# Autodesk Inventor assembly: GarageAndBracket3inchPvcPipeV02
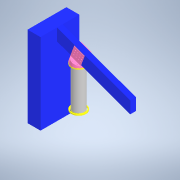
[picture p0: Inventor's stored thumbnail of the model, 180x180]
Saved by Autodesk Inventor 2022.2 (Build 262287000, 287)
## iProperties
Created: 2022-01-14
Part Number: GarageAndBracket3inchPvcPipeV02
Document SubType Name: Assembly
Designer: robst
Author: robst
## Documents named in this file (5)
- C:\git\CAD-Development\robSteele\ShapeWays\GlobalMeteorNetwork\GarageAndBracket3inchPvcPipeV02.iam
- C:\git\CAD-Development\robSteele\ShapeWays\GlobalMeteorNetwork\GarageSegment.ipt
- C:\git\CAD-Development\robSteele\ShapeWays\GlobalMeteorNetwork\bracketForGarageUpperHalfV02.ipt
- C:\git\CAD-Development\robSteele\ShapeWays\GlobalMeteorNetwork\3inPvcCap.ipt
- C:\git\CAD-Development\robSteele\ShapeWays\GlobalMeteorNetwork\3inchPvcPipe.ipt
## Components (5 placed, 4 different names)
1. GarageSegment:1 — Mate:1, Mate:2
2. bracketForGarageUpperHalfV02:1 — Mate:1, Mate:2, Insert:1
3. 3inPvcCap:1 — Mate:4, Insert:1
4. 3inchPvcPipe:1 — Mate:4, Insert:2
5. 3inPvcCap:2 — Insert:2
## Relationships (5: Mate 3, Insert 2)
- Mate:1: GarageSegment:1 ↔ bracketForGarageUpperHalfV02:1
- Mate:2: GarageSegment:1 ↔ bracketForGarageUpperHalfV02:1
- Mate:4: 3inPvcCap:1 ↔ 3inchPvcPipe:1
- Insert:1: bracketForGarageUpperHalfV02:1 ↔ 3inPvcCap:1
- Insert:2: 3inchPvcPipe:1 ↔ 3inPvcCap:2
